# Autodesk Inventor assembly: 303-dummy
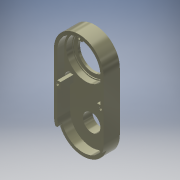
[picture p0: Inventor's stored thumbnail of the model, 180x180]
Saved by Autodesk Inventor 2018 (Build 220112000, 112)
## iProperties
Created: 2020-05-16
Part Number: 303-dummy
Document SubType Name: Assembly
Designer: Bunny320
Author: Bunny320
## Documents named in this file (3)
- C:\Users\Bunny320\Desktop\sechs\4-CAD\303-dummy.iam
- C:\Users\Bunny320\Desktop\sechs\4-CAD\303-link right-dummy down.ipt
- C:\Users\Bunny320\Desktop\sechs\4-CAD\303-link right-dummy up.ipt
## Components (2 placed, 2 different names)
1. 303-link right-dummy down:1 — Mate:1, Flush:1, Flush:2
2. 303-link right-dummy up:1 — Mate:1, Flush:1, Flush:2
## Relationships (3: Flush 2, Mate 1)
- Mate:1: 303-link right-dummy down:1 ↔ 303-link right-dummy up:1
- Flush:1: 303-link right-dummy down:1 ↔ 303-link right-dummy up:1
- Flush:2: 303-link right-dummy down:1 ↔ 303-link right-dummy up:1
